# Autodesk Inventor assembly: nozzle_v1 (laminar)
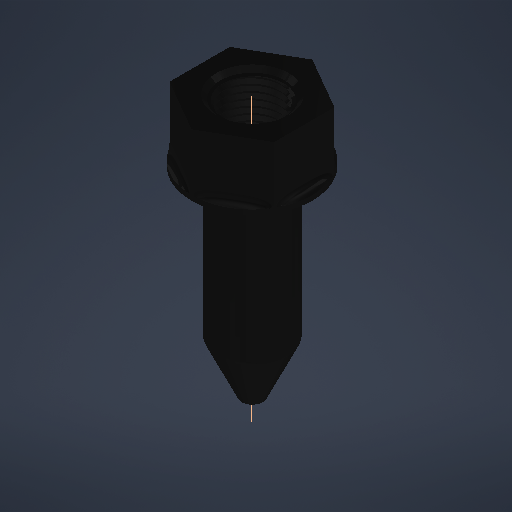
[picture p0: Inventor's stored thumbnail of the model, 512x512]
Saved by Autodesk Inventor 2026.2 (Build 302298000, 298)
## iProperties
Created: 2026-02-08
Part Number: nozzle_v1 (laminar)
Document SubType Name: Assembly
Designer: User
Author: User
## Documents named in this file (3)
- C:\Users\User\Classes\Capstone\3d\redesign but smaller\nozzle_v1 (laminar).iam
- C:\Users\User\Classes\Capstone\3d\redesign but smaller\laminar_flow.ipt
- C:\Users\User\Classes\Capstone\3d\redesign but smaller\Adapter_0_25_NPTd11_65mm_female_to_0_25_NPTd11_65mm_female.ipt
## Components (2 placed, 2 different names)
1. laminar_flow:1 — Mate:1, Mate:2, Mate:3
2. Adapter_0_25_NPTd11_65mm_female_to_0_25_NPTd11_65mm_female:1 — Mate:1, Mate:2, Mate:3
## Relationships (3: Mate 3)
- Mate:1: laminar_flow:1 ↔ Adapter_0_25_NPTd11_65mm_female_to_0_25_NPTd11_65mm_female:1
- Mate:2: laminar_flow:1 ↔ Adapter_0_25_NPTd11_65mm_female_to_0_25_NPTd11_65mm_female:1
- Mate:3: laminar_flow:1 ↔ Adapter_0_25_NPTd11_65mm_female_to_0_25_NPTd11_65mm_female:1
